# Autodesk Inventor assembly: RoboRIo
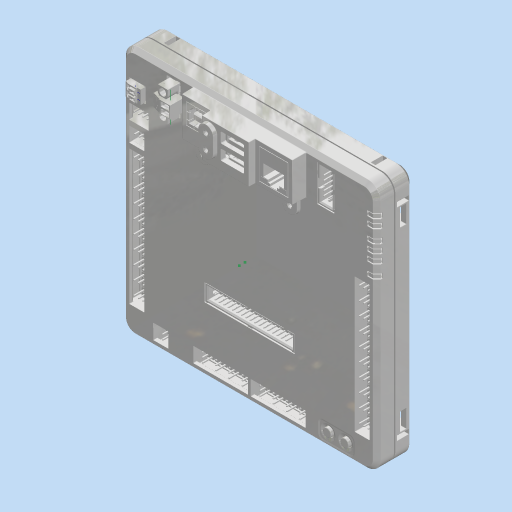
[picture p0: Inventor's stored thumbnail of the model, 512x512]
Saved by Autodesk Inventor 2023 (Build 270158000, 158)
## iProperties
Created: 2023-12-03
Part Number: RoboRIo
Document SubType Name: Assembly
Designer: Adam Arnold
Author: Adam Arnold
## Documents named in this file (3)
- J:\My Drive\1939\2_Design\2023-2024\Parts\Electronics\Logic and Control\RoboRIo.iam
- J:\My Drive\1939\2_Design\2023-2024\Parts\Electronics\Logic and Control\cd_roborio.ipt
- J:\My Drive\1939\2_Design\2023-2024\Parts\Electronics\PDH Parts\Can Block.ipt
## Components (3 placed, 2 different names)
1. cd_roborio:1 — Flush:1, Flush:2, Flush:3, Flush:4, Flush:5, Flush:6
2. Can Block:1 — Flush:1, Flush:5, Flush:6
3. Can Block:2 — Flush:2, Flush:3, Flush:4
## Relationships (6: Flush 6)
- Flush:1: cd_roborio:1 ↔ Can Block:1
- Flush:2: cd_roborio:1 ↔ Can Block:2
- Flush:3: cd_roborio:1 ↔ Can Block:2
- Flush:4: cd_roborio:1 ↔ Can Block:2
- Flush:5: cd_roborio:1 ↔ Can Block:1
- Flush:6: cd_roborio:1 ↔ Can Block:1
